# Autodesk Inventor assembly: Chwytak
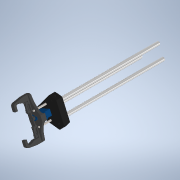
[picture p0: Inventor's stored thumbnail of the model, 180x180]
Saved by Autodesk Inventor 2021 (Build 250183000, 183)
## iProperties
Created: 2021-07-30
Part Number: Chwytak
Document SubType Name: Assembly
Designer: Janusz
Author: Janusz
Revision Number: ANY
## Documents named in this file (8)
- D:\ROBOT\Chwytak.iam
- D:\ROBOT\Zalepka_osi_Z.iam
- D:\ROBOT\Chwytak_liniowy_kr¢tkie.iam
- D:\ROBOT\ISO 10642 - M4 x 40 - 20N_ISO 10642 - M4 x 40 - 20N.ipt
- D:\ROBOT\bering_osiowy.ipt
- D:\ROBOT\podk³adka_ciskowa.ipt
- D:\ROBOT\rod_8mm_200.ipt
- D:\ROBOT\rod_8mm_250.ipt
## Components (10 placed, 10 different names)
1. Zalepka_osi_Z_7 [sub-assembly] — Zestawiające:1, Zestawiające:2, Zestawiające:3, Zestawiające:4, Zestawiające:5, Zestawiające:6, Zestawiające:7, Sztywne:1, Zestawiające:8, Zestawiające:9, Zestawiające:10
2. Chwytak_liniowy_kr¢tkie_8 [sub-assembly] — Zestawiające:6, Zestawiające:7, Zestawiające:10
3. ISO 10642 - M4 x 40 - 20N_ISO 10642 - M4 x 40 - 20N_9 — Zestawiające:9
4. ISO 10642 - M4 x 40 - 20N_ISO 10642 - M4 x 40 - 20N_10 — Zestawiające:8
5. bering_osiowy_11
6. bering_osiowy_12
7. podk³adka_ciskowa_13
8. rod_8mm_200_14 — Zestawiające:3, Sztywne:1
9. rod_8mm_250_15 — Zestawiające:2, Zestawiające:5
10. rod_8mm_250_16 — Zestawiające:1, Zestawiające:4
## Relationships (11: Mate 10, WeldJoint 1)
- Zestawiające:1 [Mate]: Zalepka_osi_Z_7 ↔ rod_8mm_250_16
- Zestawiające:2 [Mate]: Zalepka_osi_Z_7 ↔ rod_8mm_250_15
- Zestawiające:3 [Mate]: Zalepka_osi_Z_7 ↔ rod_8mm_200_14
- Zestawiające:4 [Mate]: Zalepka_osi_Z_7 ↔ rod_8mm_250_16
- Zestawiające:5 [Mate]: Zalepka_osi_Z_7 ↔ rod_8mm_250_15
- Zestawiające:6 [Mate]: Zalepka_osi_Z_7 ↔ Chwytak_liniowy_kr¢tkie_8
- Zestawiające:7 [Mate]: Zalepka_osi_Z_7 ↔ Chwytak_liniowy_kr¢tkie_8
- Sztywne:1 [WeldJoint]: Zalepka_osi_Z_7 ↔ rod_8mm_200_14
- Zestawiające:8 [Mate]: Zalepka_osi_Z_7 ↔ ISO 10642 - M4 x 40 - 20N_ISO 10642 - M4 x 40 - 20N_10
- Zestawiające:9 [Mate]: Zalepka_osi_Z_7 ↔ ISO 10642 - M4 x 40 - 20N_ISO 10642 - M4 x 40 - 20N_9
- Zestawiające:10 [Mate]: Zalepka_osi_Z_7 ↔ Chwytak_liniowy_kr¢tkie_8
